# Autodesk Inventor assembly: Assembly146-01
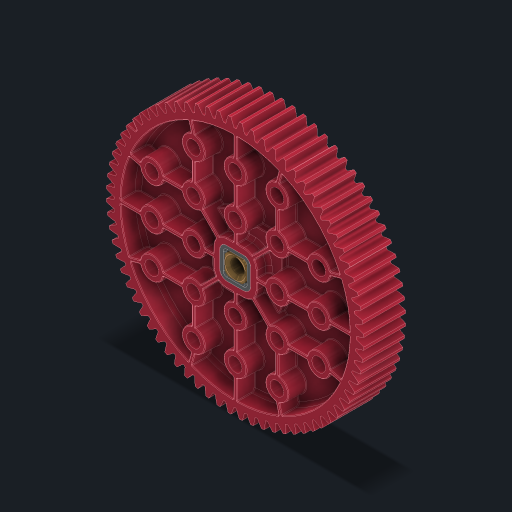
[picture p0: Inventor's stored thumbnail of the model, 512x512]
Saved by Autodesk Inventor 2024 (Build 280153000, 153)
## iProperties
Created: 2022-08-02
Part Number: Assembly146-01
Document SubType Name: Assembly
Designer: ylu12
Author: ylu12
## Documents named in this file (4)
- D:\vex_robotics\hardware\cad\VEX-CAD-Inventor-main\Motion\Gears\HS Gear\HS 72T Gear, Circle.iam
- D:\vex_robotics\hardware\cad\VEX-CAD-Inventor-main\Motion\HS Shaft Adapter Circle.ipt
- D:\vex_robotics\hardware\cad\VEX-CAD-Inventor-main\Motion\Gears\Reference Files\HS 72T Gear, No Insert.ipt
- D:\vex_robotics\hardware\cad\VEX-CAD-Inventor-main\Motion\Gears\HS Gear.iam
## Components (2 placed, 2 different names)
1. Circle — Mate:1, Mate:2, Flush:1
2. 72T — Flush:8, Mate:15, Mate:16
## Relationships (6: Mate 4, Flush 2)
- Mate:1: Circle
- Mate:2: Circle
- Flush:1 (6.35 mm): Circle
- Flush:8: 72T
- Mate:15: 72T
- Mate:16: 72T
